# Autodesk Inventor assembly: 3.25" Omni-Directional Wheel, Square Insert
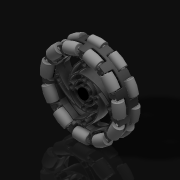
[picture p0: Inventor's stored thumbnail of the model, 180x180]
Saved by Autodesk Inventor 2021 (Build 250183000, 183)
## iProperties
Created: 2014-06-25
Document SubType Name: Assembly
Designer: Jordan Kiesel
Vendor: VEX Robotics, Inc.
Mass: 65.0215 g
Surface Area: 582.822 cm^2
Volume: 43.4914 cm^3
Density: 1.49504 g/cm^3
Company: Bots 'n' Stuff
Author: Jordan Kiesel
Title: 3.25" Omni-Directional Wheel, Square Insert
## Documents named in this file (3)
- E:\VEX Library\Motion\Wheels _ Rollers\3.25 Omni, Square Insert.iam
- E:\VEX Library\Motion\Wheels _ Rollers\Reference Parts\3.25_ Omni-Directional Wheels\3.25_ Omni-Directional Wheel.iam
- E:\VEX Library\Motion\Reference Parts\High Strength Square Gear Insert.ipt
## Components (3 placed, 2 different names)
1. 3.25_ Omni-Directional Wheel:1 [sub-assembly] — Mate:1, Mate:2, Mate:3, Mate:4, Mate:5, Mate:6
2. High Strength Square Gear Insert:1 — Mate:1, Mate:2, Mate:3
3. High Strength Square Gear Insert:2 — Mate:4, Mate:5, Mate:6
## Relationships (6: Mate 6)
- Mate:1 (0.0254 mm): 3.25_ Omni-Directional Wheel:1 ↔ High Strength Square Gear Insert:1
- Mate:2 (0.0254 mm): 3.25_ Omni-Directional Wheel:1 ↔ High Strength Square Gear Insert:1
- Mate:3: 3.25_ Omni-Directional Wheel:1 ↔ High Strength Square Gear Insert:1
- Mate:4 (0.0254 mm): 3.25_ Omni-Directional Wheel:1 ↔ High Strength Square Gear Insert:2
- Mate:5 (0.0254 mm): 3.25_ Omni-Directional Wheel:1 ↔ High Strength Square Gear Insert:2
- Mate:6: 3.25_ Omni-Directional Wheel:1 ↔ High Strength Square Gear Insert:2
